# Autodesk Inventor assembly: Shoulder
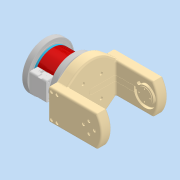
[picture p0: Inventor's stored thumbnail of the model, 180x180]
Saved by Autodesk Inventor 2020.2 (Build 242310000, 310)
## iProperties
Created: 2020-02-11
Part Number: Shoulder
Document SubType Name: Assembly
Designer: JochenAlt
Author: JochenAlt
## Documents named in this file (4)
- D:\Projects\MiniBot\CAD\Shoulder.iam
- D:\Projects\MiniBot\CAD\extern\bearings\65x85x10\61813-2RS1.iam
- D:\Projects\MiniBot\CAD\extern\Herkulex\Herkulex DRS-040x.ipt
- D:\Projects\MiniBot\CAD\Shoulder.ipt
## Components (4 placed, 3 different names)
1. 61813-2RS1:1 [sub-assembly] — Passend:7, Passend:10
2. 61813-2RS1:2 [sub-assembly] — Passend:8, Passend:11
3. Herkulex DRS-040x:1 — Passend:9, Passend:13, Winkel:1
4. Shoulder:1 — Passend:7, Passend:8, Passend:9, Passend:10, Passend:11, Passend:13, Winkel:1
## Relationships (7: Mate 6, Angle 1)
- Passend:7 [Mate]: 61813-2RS1:1 ↔ Shoulder:1
- Passend:8 [Mate]: 61813-2RS1:2 ↔ Shoulder:1
- Passend:9 [Mate]: Herkulex DRS-040x:1 ↔ Shoulder:1
- Passend:10 [Mate]: 61813-2RS1:1 ↔ Shoulder:1
- Passend:11 [Mate]: 61813-2RS1:2 ↔ Shoulder:1
- Passend:13 [Mate]: Herkulex DRS-040x:1 ↔ Shoulder:1
- Winkel:1 [Angle] (-90 deg): Herkulex DRS-040x:1 ↔ Shoulder:1
